# Autodesk Inventor assembly: 6P 8T Sprocket, No Insert_mirrored
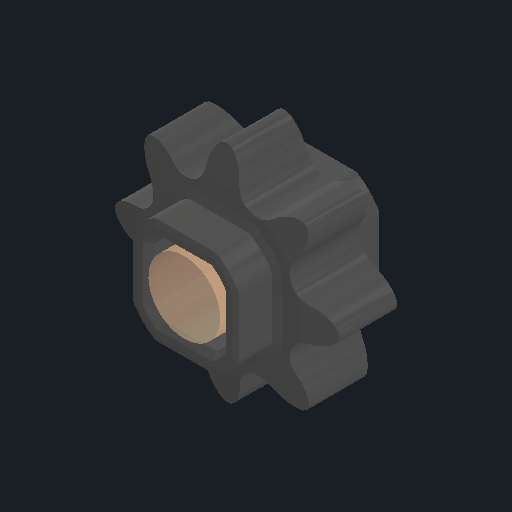
[picture p0: Inventor's stored thumbnail of the model, 512x512]
Saved by Autodesk Inventor 2025 (Build 290162000, 162)
## iProperties
Created: 2022-08-02
Part Number: 6P 8T Sprocket, No Insert_mirrored
Document SubType Name: Assembly
Designer: Averey Ku
Author: ylu12
## Documents named in this file (2)
- D:\vex_robotics_high_stakes\hardware\cad\EARLY_SEASON\tower\mirored_parts\6P 8T Sprocket, No Insert_mirrored.iam
- D:\vex_robotics_high_stakes\hardware\cad\EARLY_SEASON\tower\mirored_parts\6P 8T Sprocket_mirrored.ipt
## Components (1 placed, 1 different names)
1. 6P 8T Sprocket_mirrored:1 — Flush:3, Mate:6, Mate:5
## Relationships (3: Mate 2, Flush 1)
- Flush:3: 6P 8T Sprocket_mirrored:1
- Mate:6: 6P 8T Sprocket_mirrored:1
- Mate:5: 6P 8T Sprocket_mirrored:1
